# Autodesk Inventor assembly: valve driver
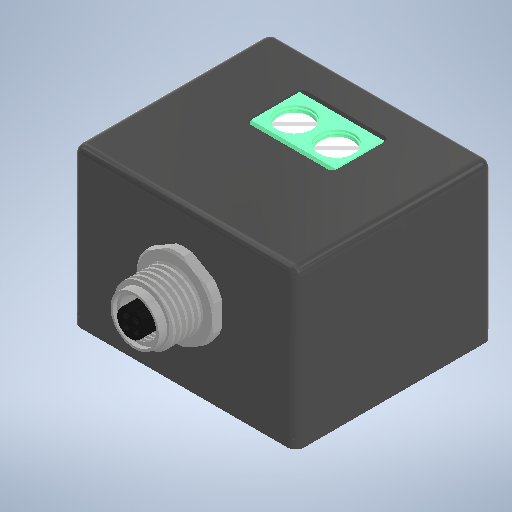
[picture p0: Inventor's stored thumbnail of the model, 512x512]
Saved by Autodesk Inventor 2025.4 (Build 294407000, 407)
## iProperties
Created: 2025-05-14
Part Number: valve driver
Document SubType Name: Assembly
Designer: Yuhsuan Chen
Author: Yuhsuan Chen
## Documents named in this file (4)
- C:\Users\Yuhsuan Chen\Desktop\github\fablabs-valve-driver\mCAD\valve driver master.iam
- C:\Users\Yuhsuan Chen\Desktop\github\fablabs-valve-driver\mCAD\PCBA\valve_driver.iam
- C:\Users\Yuhsuan Chen\Desktop\github\fablabs-valve-driver\mCAD\bottom cover.ipt
- C:\Users\Yuhsuan Chen\Desktop\github\fablabs-valve-driver\mCAD\top cover.ipt
## Components (3 placed, 3 different names)
1. valve_driver:2 [sub-assembly] — Mate:1, Mate:2, Flush:1, Mate:9
2. bottom cover:1 — Mate:7, Flush:4, Mate:9, Mate:10
3. top cover:1 — Mate:6, Flush:5, Mate:10
## Relationships (9: Mate 6, Flush 3)
- Mate:1: valve_driver:2
- Mate:2: valve_driver:2
- Flush:1: valve_driver:2
- Mate:6 (-0.55 mm): top cover:1
- Mate:7: bottom cover:1
- Flush:4: bottom cover:1
- Flush:5: top cover:1
- Mate:9: valve_driver:2 ↔ bottom cover:1
- Mate:10: bottom cover:1 ↔ top cover:1
